# Autodesk Inventor assembly: main
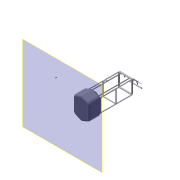
[picture p0: Inventor's stored thumbnail of the model, 180x180]
Saved by Autodesk Inventor 2014 SP1 (Build 180222100, 222)
## iProperties
Created: 2015-02-04
Part Number: main
Document SubType Name: Assembly
Designer: Simen
Author: Simen
## Documents named in this file (5)
- C:\Users\Simen\Documents\git\Eit\skjellet\main.iam
- C:\Users\Simen\Documents\git\Eit\skjellet\base.iam
- C:\Users\Simen\Documents\git\Eit\skjellet\skellett.iam
- C:\Users\Simen\Documents\git\Eit\skjellet\Head.iam
- C:\Users\Simen\Documents\git\Eit\skjellet\Head2.iam
## Components (4 placed, 4 different names)
1. base:1 [sub-assembly] — Mate:5, Flush:16, Mate:7, Mate:8, Mate:9, Mate:10
2. skellett:1 [sub-assembly] — Mate:5, Flush:16, Flush:20, Flush:21, Mate:9, Mate:10, Flush:22, Flush:23
3. Head:1 [sub-assembly] — Flush:20, Flush:21
4. Head2:1 [sub-assembly] — Flush:22, Flush:23
## Relationships (10: Mate 5, Flush 5)
- Mate:5: base:1 ↔ skellett:1
- Flush:16 (6 mm): base:1 ↔ skellett:1
- Mate:7: base:1
- Mate:8: base:1
- Flush:20: skellett:1 ↔ Head:1
- Flush:21: skellett:1 ↔ Head:1
- Mate:9: base:1 ↔ skellett:1
- Mate:10 (20 mm): base:1 ↔ skellett:1
- Flush:22: skellett:1 ↔ Head2:1
- Flush:23: skellett:1 ↔ Head2:1
